# Autodesk Inventor assembly: AssemblyBench
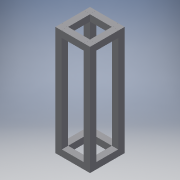
[picture p0: Inventor's stored thumbnail of the model, 180x180]
Saved by Autodesk Inventor 2017 (Build 210142000, 142)
## iProperties
Created: 2019-07-06
Part Number: AssemblyBench
Document SubType Name: Assembly
Designer: Ole Simmering
Author: Ole Simmering
## Documents named in this file (4)
- C:\Users\Ole Simmering\Documents\GitHub\3D_modeling\Guillotine\AssemblyBench.iam
- C:\Users\Ole Simmering\Documents\GitHub\3D_modeling\Guillotine\4x4x5feet.ipt
- C:\Users\Ole Simmering\Documents\GitHub\3D_modeling\Guillotine\4ix4ix6i.ipt
- C:\Users\Ole Simmering\Documents\GitHub\3D_modeling\Guillotine\4ix4ix6i_MIR.ipt
## Components (12 placed, 3 different names)
1. 4x4x5feet:1 — Mate:2, Flush:3, Flush:4, Symmetry:1
2. 4x4x5feet:2 — Mate:1, Flush:1, Flush:2, Mate:3, Flush:5, Flush:6
3. 4x4x5feet:3 — Mate:6, Flush:11, Flush:12, Mate:7, Flush:13, Flush:14
4. 4x4x5feet:4 — Mate:4, Flush:7, Flush:8, Mate:5, Flush:9, Flush:10, Symmetry:1
5. 4ix4ix6i:5 — Mate:3, Flush:5, Flush:6, Mate:4, Flush:7, Flush:8
6. 4ix4ix6i:6 — Mate:7, Flush:13, Flush:14
7. 4ix4ix6i:7 — Mate:5, Flush:9, Flush:10, Mate:6, Flush:11, Flush:12
8. 4ix4ix6i:8 — Mate:1, Flush:1, Flush:2, Mate:2, Flush:3, Flush:4
9. 4ix4ix6i_MIR:1
10. 4ix4ix6i_MIR:2
11. 4ix4ix6i_MIR:3
12. 4ix4ix6i_MIR:4
## Relationships (22: Flush 14, Mate 7, Symmetry 1)
- Mate:1: 4x4x5feet:2 ↔ 4ix4ix6i:8
- Flush:1: 4x4x5feet:2 ↔ 4ix4ix6i:8
- Flush:2: 4x4x5feet:2 ↔ 4ix4ix6i:8
- Mate:2: 4x4x5feet:1 ↔ 4ix4ix6i:8
- Flush:3: 4x4x5feet:1 ↔ 4ix4ix6i:8
- Flush:4: 4x4x5feet:1 ↔ 4ix4ix6i:8
- Mate:3: 4x4x5feet:2 ↔ 4ix4ix6i:5
- Flush:5: 4x4x5feet:2 ↔ 4ix4ix6i:5
- Flush:6: 4x4x5feet:2 ↔ 4ix4ix6i:5
- Mate:4: 4x4x5feet:4 ↔ 4ix4ix6i:5
- Flush:7: 4x4x5feet:4 ↔ 4ix4ix6i:5
- Flush:8: 4x4x5feet:4 ↔ 4ix4ix6i:5
- Mate:5: 4x4x5feet:4 ↔ 4ix4ix6i:7
- Flush:9: 4x4x5feet:4 ↔ 4ix4ix6i:7
- Flush:10: 4x4x5feet:4 ↔ 4ix4ix6i:7
- Mate:6: 4x4x5feet:3 ↔ 4ix4ix6i:7
- Flush:11: 4x4x5feet:3 ↔ 4ix4ix6i:7
- Flush:12: 4x4x5feet:3 ↔ 4ix4ix6i:7
- Mate:7: 4x4x5feet:3 ↔ 4ix4ix6i:6
- Flush:13: 4x4x5feet:3 ↔ 4ix4ix6i:6
- Flush:14: 4x4x5feet:3 ↔ 4ix4ix6i:6
- Symmetry:1: 4x4x5feet:1 ↔ 4x4x5feet:4
